# Autodesk Inventor assembly: sindouki_assem v1
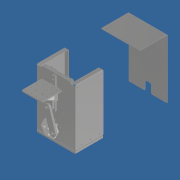
[picture p0: Inventor's stored thumbnail of the model, 180x180]
Saved by Autodesk Inventor 2020 (Build 240168000, 168)
## iProperties
Created: 2021-08-17
Part Number: sindouki_assem v1
Document SubType Name: Assembly
Designer: ken113
Sending System: Autodesk Translation Framework v10.9.0.1377
Preprocessor: ST-DEVELOPER v18.1
Title: D:/Downloads/sindouki_assem v1.step
## Documents named in this file (21)
- D:\Document\Github\Vibration_Generator\Parts\Sample\sindouki_assem v1.iam
- D:\Document\Github\Vibration_Generator\Parts\Sample\A1816_F v1.ipt
- D:\Document\Github\Vibration_Generator\Parts\Sample\SOL5M8F v1.ipt
- D:\Document\Github\Vibration_Generator\Parts\Sample\part1 v1.ipt
- D:\Document\Github\Vibration_Generator\Parts\Sample\part2 v1.ipt
- D:\Document\Github\Vibration_Generator\Parts\Sample\MCOC30-12-14 v1.iam
- D:\Document\Github\Vibration_Generator\Parts\Sample\BGRAB6001ZZ v1.iam
- D:\Document\Github\Vibration_Generator\Parts\Sample\80W-12 v1.ipt
- D:\Document\Github\Vibration_Generator\Parts\Sample\part4 v1.ipt
- D:\Document\Github\Vibration_Generator\Parts\Sample\part5 v1.ipt
- D:\Document\Github\Vibration_Generator\Parts\Sample\SXRL24-150 v1.iam
- D:\Document\Github\Vibration_Generator\Parts\Sample\100_100 v1.ipt
- D:\Document\Github\Vibration_Generator\Parts\Sample\main_cover v1.ipt
- D:\Document\Github\Vibration_Generator\Parts\Sample\HFS6-3030-272 v1.ipt
- D:\Document\Github\Vibration_Generator\Parts\Sample\SFL6800ZZ v1.ipt
- D:\Document\Github\Vibration_Generator\Parts\Sample\PACK10-CIMRS12-15-0.5 v1.ipt
- D:\Document\Github\Vibration_Generator\Parts\Sample\SSTHR12-MB v1.iam
- D:\Document\Github\Vibration_Generator\Parts\Sample\PSSFG12-53-RC12 v1.ipt
- D:\Document\Github\Vibration_Generator\Parts\Meviy\Flange.ipt
- D:\Document\Github\Vibration_Generator\Parts\Meviy\Plate_Angle.ipt
- D:\Document\Github\Vibration_Generator\Parts\MISUMI\FSSFJBF-D10-L20-M5-U3_Autodesk_Inventor_2020_20210817 (2)\FSSFJBF-D10-L20-M5-U3.ipt
## Components (28 placed, 20 different names)
1. A1816_F v1:1 — 挿入:12, メイト:7
2. SOL5M8F v1:1 — 挿入:15, 挿入:16
3. part1 v1:2 — 挿入:17, 挿入:18, メイト:8, メイト:9, メイト:11, メイト:12, メイト:14
4. part2 v1:1 — 挿入:13, 挿入:14, 角度:1, 挿入:15, 挿入:16, 挿入:17, 挿入:18
5. MCOC30-12-14 v1:1 [sub-assembly] — 挿入:12
6. BGRAB6001ZZ v1:1 [sub-assembly] — メイト:2, メイト:3, メイト:7, メイト:8, メイト:9
7. 80W-12 v1:2
8. part4 v1:1 — 挿入:10, 挿入:11, 挿入:21, メイト:10, フラッシュ:2, 挿入:23, 挿入:25, 挿入:26
9. part5 v1:1 — 挿入:1, 挿入:2, 挿入:5, 挿入:6
10. SXRL24-150 v1:1 [sub-assembly] — 挿入:10, 挿入:11, メイト:11, メイト:12, メイト:14
11. 100*100 v1:1 — 挿入:22, メイト:13
12. main_cover v1:1
13. HFS6-3030-272 v1:1 — 挿入:13, フラッシュ:1
14. HFS6-3030-272 v1:2 — 挿入:14, 角度:1, フラッシュ:1
15. SFL6800ZZ v1:2 — 挿入:2, 挿入:3
16. SFL6800ZZ v1:4 — 挿入:6, 挿入:8
17. SFL6800ZZ v1:6 — 挿入:5, 挿入:7
18. SFL6800ZZ v1:7 — 挿入:1, 挿入:4, メイト:6
19. PACK10-CIMRS12-15-0.5 v1:1 — 挿入:8, 挿入:21
20. PACK10-CIMRS12-15-0.5 v1:2 — 挿入:3, メイト:5
21. PACK10-CIMRS12-15-0.5 v1:3 — 挿入:7
22. PACK10-CIMRS12-15-0.5 v1:4 — 挿入:4
23. SSTHR12-MB v1:1 [sub-assembly] — 挿入:19, 挿入:20, メイト:4
24. PSSFG12-53-RC12 v1:1 — メイト:3, 挿入:19
25. Flange:1 — メイト:2, 挿入:20, メイト:4, メイト:5, メイト:6, 挿入:24
26. Plate_Angle:1 — メイト:10, フラッシュ:2, 挿入:22, メイト:13, 挿入:25, 挿入:26
27. FSSFJBF-D10-L20-M5-U3:1 — 挿入:24
28. FSSFJBF-D10-L20-M5-U3:2 — 挿入:23
## Relationships (41: Insert 25, Mate 13, Flush 2, Angle 1)
- 挿入:1 [Insert]: part5 v1:1 ↔ SFL6800ZZ v1:7
- 挿入:2 [Insert]: part5 v1:1 ↔ SFL6800ZZ v1:2
- 挿入:3 [Insert]: SFL6800ZZ v1:2 ↔ PACK10-CIMRS12-15-0.5 v1:2
- 挿入:4 [Insert]: SFL6800ZZ v1:7 ↔ PACK10-CIMRS12-15-0.5 v1:4
- 挿入:5 [Insert]: part5 v1:1 ↔ SFL6800ZZ v1:6
- 挿入:6 [Insert]: part5 v1:1 ↔ SFL6800ZZ v1:4
- 挿入:7 [Insert]: SFL6800ZZ v1:6 ↔ PACK10-CIMRS12-15-0.5 v1:3
- 挿入:8 [Insert]: SFL6800ZZ v1:4 ↔ PACK10-CIMRS12-15-0.5 v1:1
- 挿入:10 [Insert]: part4 v1:1 ↔ SXRL24-150 v1:1
- 挿入:11 [Insert]: part4 v1:1 ↔ SXRL24-150 v1:1
- メイト:2 [Mate]: BGRAB6001ZZ v1:1 ↔ Flange:1
- 挿入:12 [Insert]: A1816_F v1:1 ↔ MCOC30-12-14 v1:1
- 挿入:13 [Insert]: part2 v1:1 ↔ HFS6-3030-272 v1:1
- 挿入:14 [Insert]: part2 v1:1 ↔ HFS6-3030-272 v1:2
- 角度:1 [Angle] (0 deg): part2 v1:1 ↔ HFS6-3030-272 v1:2
- フラッシュ:1 [Flush]: HFS6-3030-272 v1:1 ↔ HFS6-3030-272 v1:2
- 挿入:15 [Insert]: SOL5M8F v1:1 ↔ part2 v1:1
- 挿入:16 [Insert]: SOL5M8F v1:1 ↔ part2 v1:1
- 挿入:17 [Insert]: part1 v1:2 ↔ part2 v1:1
- 挿入:18 [Insert]: part1 v1:2 ↔ part2 v1:1
- メイト:3 [Mate]: BGRAB6001ZZ v1:1 ↔ PSSFG12-53-RC12 v1:1
- 挿入:19 [Insert]: SSTHR12-MB v1:1 ↔ PSSFG12-53-RC12 v1:1
- 挿入:20 [Insert]: SSTHR12-MB v1:1 ↔ Flange:1
- メイト:4 [Mate]: SSTHR12-MB v1:1 ↔ Flange:1
- メイト:5 [Mate]: PACK10-CIMRS12-15-0.5 v1:2 ↔ Flange:1
- メイト:6 [Mate]: SFL6800ZZ v1:7 ↔ Flange:1
- 挿入:21 [Insert]: part4 v1:1 ↔ PACK10-CIMRS12-15-0.5 v1:1
- メイト:7 [Mate]: A1816_F v1:1 ↔ BGRAB6001ZZ v1:1
- メイト:8 [Mate]: part1 v1:2 ↔ BGRAB6001ZZ v1:1
- メイト:9 [Mate]: part1 v1:2 ↔ BGRAB6001ZZ v1:1
- メイト:10 [Mate]: part4 v1:1 ↔ Plate_Angle:1
- フラッシュ:2 [Flush]: part4 v1:1 ↔ Plate_Angle:1
- メイト:11 [Mate]: part1 v1:2 ↔ SXRL24-150 v1:1
- メイト:12 [Mate]: part1 v1:2 ↔ SXRL24-150 v1:1
- 挿入:22 [Insert]: 100*100 v1:1 ↔ Plate_Angle:1
- メイト:13 [Mate]: 100*100 v1:1 ↔ Plate_Angle:1
- 挿入:23 [Insert]: part4 v1:1 ↔ FSSFJBF-D10-L20-M5-U3:2
- 挿入:24 [Insert]: Flange:1 ↔ FSSFJBF-D10-L20-M5-U3:1
- 挿入:25 [Insert]: part4 v1:1 ↔ Plate_Angle:1
- 挿入:26 [Insert]: part4 v1:1 ↔ Plate_Angle:1
- メイト:14 [Mate]: part1 v1:2 ↔ SXRL24-150 v1:1
